# Autodesk Inventor assembly: U2D2 and Power Board Assembly
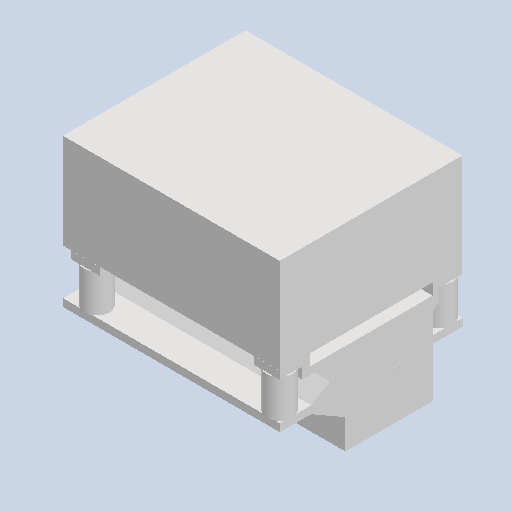
[picture p0: Inventor's stored thumbnail of the model, 512x512]
Saved by Autodesk Inventor 2022 (Build 260153000, 153)
## iProperties
Created: 2021-09-20
Part Number: U2D2 and Power Board Assembly
Document SubType Name: Assembly
Designer: kylem
Author: kylem
## Documents named in this file (5)
- C:\Users\kylem\OneDrive\Documents\GitHub\IMML_Contactile_Gripper_Hardware\U2D2 and Power Board Assembly.iam
- C:\Users\kylem\OneDrive\Documents\GitHub\IMML_Contactile_Gripper_Hardware\U2D2.ipt
- C:\Users\kylem\OneDrive\Documents\GitHub\IMML_Contactile_Gripper_Hardware\U2D2PHB_Board.ipt
- C:\Users\kylem\OneDrive\Documents\GitHub\IMML_Contactile_Gripper_Hardware\U2D2 Plate.ipt
- C:\Users\kylem\OneDrive\Documents\GitHub\IMML_Contactile_Gripper_Hardware\U2D2 Plate v2.ipt
## Components (4 placed, 4 different names)
1. U2D2:1 — Flush:1, Angle:1, Flush:2, Mate:1
2. U2D2PHB_Board:1 — Flush:1, Angle:1, Flush:2, Mate:1, Mate:2, Flush:3, Mate:3, Mate:4, Mate:5, Angle:2
3. U2D2 Plate:1 — Mate:2, Flush:3, Mate:3
4. U2D2 Plate v2:1 — Mate:4, Mate:5, Angle:2
## Relationships (10: Mate 5, Flush 3, Angle 2)
- Flush:1: U2D2:1 ↔ U2D2PHB_Board:1
- Angle:1 (0 deg): U2D2:1 ↔ U2D2PHB_Board:1
- Flush:2: U2D2:1 ↔ U2D2PHB_Board:1
- Mate:1 (5 mm): U2D2:1 ↔ U2D2PHB_Board:1
- Mate:2: U2D2PHB_Board:1 ↔ U2D2 Plate:1
- Flush:3: U2D2PHB_Board:1 ↔ U2D2 Plate:1
- Mate:3: U2D2PHB_Board:1 ↔ U2D2 Plate:1
- Mate:4: U2D2PHB_Board:1 ↔ U2D2 Plate v2:1
- Mate:5: U2D2PHB_Board:1 ↔ U2D2 Plate v2:1
- Angle:2 (0 deg): U2D2PHB_Board:1 ↔ U2D2 Plate v2:1
